# Autodesk Inventor assembly: Assembly_neje_slide_plate
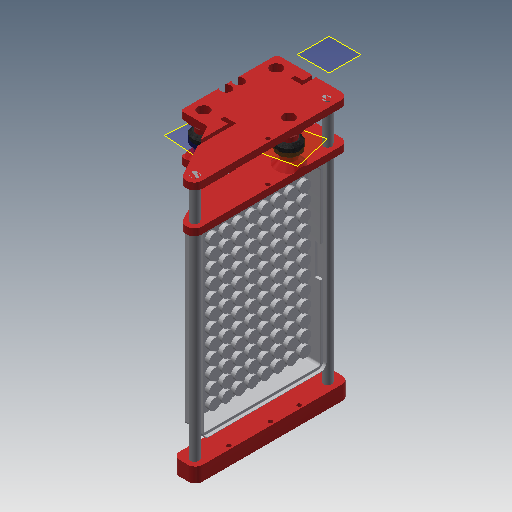
[picture p0: Inventor's stored thumbnail of the model, 512x512]
Saved by Autodesk Inventor 2019.4 (Build 234330000, 330)
## iProperties
Created: 2021-04-08
Part Number: Assembly_neje_slide_plate
Document SubType Name: Assembly
Designer: diederichbenedict
Mass: 112.697 g
Surface Area: 1375.99 cm^2
Volume: 112.697 cm^3
Density: 1 g/cm^3
Author: diederichbenedict
## Documents named in this file (7)
- C:\Users\diederichbenedict\Dropbox\Dokumente\Promotion\PROJECTS\UC2\02_CAD\INVENTOR\uc2_v3\Assembly_neje_slide_plate.iam
- C:\Users\diederichbenedict\Dropbox\Dokumente\Promotion\PROJECTS\UC2\02_CAD\INVENTOR\uc2_v3\Neje_Base_Slide_y_20mmrod.ipt
- C:\Users\diederichbenedict\Dropbox\Dokumente\Promotion\PROJECTS\UC2\02_CAD\INVENTOR\uc2_v3\Neje_Base_Slide_y_20mmrod_R11.ipt
- C:\Users\diederichbenedict\Dropbox\Dokumente\Promotion\PROJECTS\UC2\02_CAD\INVENTOR\uc2_v3\Neje_Base_Slide_y_stop.ipt
- C:\Users\diederichbenedict\Dropbox\Dokumente\Promotion\PROJECTS\UC2\02_CAD\INVENTOR\uc2_v3\00_Thorlabs_Rod_6mm.ipt
- C:\Users\diederichbenedict\Dropbox\Dokumente\Promotion\PROJECTS\UC2\02_CAD\INVENTOR\uc2_v3\00_MTP_96-welplate.ipt
- C:\Users\diederichbenedict\Dropbox\Dokumente\Promotion\PROJECTS\UC2\02_CAD\INVENTOR\uc2_v3\Neje_Rolls_small.ipt
## Components (9 placed, 6 different names)
1. Neje_Rolls_small:2
2. Neje_Rolls_small:1 — Insert:16
3. Neje_Rolls_small:3
4. Neje_Base_Slide_y_20mmrod:1 — Angle:1, Mate:5
5. 00_Thorlabs_Rod_6mm:1 — Insert:19
6. Neje_Base_Slide_y_20mmrod_R11:1 — Insert:16, Angle:1, Mate:5, Mate:6
7. 00_Thorlabs_Rod_6mm:2 — Insert:18
8. Neje_Base_Slide_y_stop:1 — Insert:18, Insert:19, Flush:1, Flush:2
9. 00_MTP_96-welplate:1 — Flush:1, Flush:2, Mate:6
## Relationships (11: Insert 6, Mate 2, Flush 2, Angle 1)
- [Insert]: Neje_Rolls_small:2 ↔ Neje_Base_Slide_y_20mmrod:1
- [Insert]: Neje_Rolls_small:1 ↔ Neje_Base_Slide_y_20mmrod:1
- [Insert]: Neje_Rolls_small:3 ↔ Neje_Base_Slide_y_20mmrod:1
- Insert:16: Neje_Rolls_small:1 ↔ Neje_Base_Slide_y_20mmrod_R11:1
- Angle:1 (180 deg): Neje_Base_Slide_y_20mmrod:1 ↔ Neje_Base_Slide_y_20mmrod_R11:1
- Mate:5: Neje_Base_Slide_y_20mmrod:1 ↔ Neje_Base_Slide_y_20mmrod_R11:1
- Insert:18: 00_Thorlabs_Rod_6mm:2 ↔ Neje_Base_Slide_y_stop:1
- Insert:19: 00_Thorlabs_Rod_6mm:1 ↔ Neje_Base_Slide_y_stop:1
- Flush:1 (9 mm): Neje_Base_Slide_y_stop:1 ↔ 00_MTP_96-welplate:1
- Flush:2 (11.5 mm): Neje_Base_Slide_y_stop:1 ↔ 00_MTP_96-welplate:1
- Mate:6: Neje_Base_Slide_y_20mmrod_R11:1 ↔ 00_MTP_96-welplate:1
